# Autodesk Inventor assembly: Mold Design1_Part1_PZ
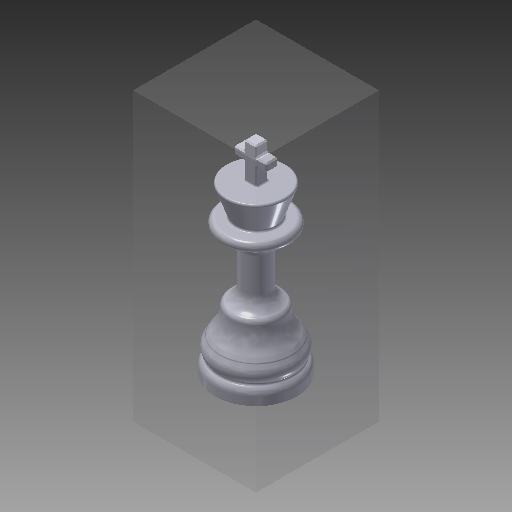
[picture p0: Inventor's stored thumbnail of the model, 512x512]
Saved by Autodesk Inventor 2018 (Build 220112000, 112)
## iProperties
Created: 2017-12-19
Part Number: Mold Design1_Part1_PZ
Document SubType Name: Assembly
Designer: 238438
Author: 238438
## Documents named in this file (3)
- P:\ied\chess\Mold Design1_Part1_PZ.iam
- P:\ied\chess\Mold Design1_Part1_MP.ipt
- P:\ied\chess\Mold Design1_Part1_WP.ipt
## Components (2 placed, 2 different names)
1. Mold Design1_Part1_MP:1 — Flush:1, Flush:2, Flush:3, Flush:4, Flush:5, Flush:6
2. Mold Design1_Part1_WP:1 — Flush:4, Flush:5, Flush:6
## Relationships (6: Flush 6)
- Flush:1: Mold Design1_Part1_MP:1
- Flush:2: Mold Design1_Part1_MP:1
- Flush:3: Mold Design1_Part1_MP:1
- Flush:4: Mold Design1_Part1_MP:1 ↔ Mold Design1_Part1_WP:1
- Flush:5: Mold Design1_Part1_MP:1 ↔ Mold Design1_Part1_WP:1
- Flush:6: Mold Design1_Part1_MP:1 ↔ Mold Design1_Part1_WP:1
